# Autodesk Inventor assembly: GFRP_T2_01
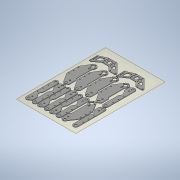
[picture p0: Inventor's stored thumbnail of the model, 180x180]
Saved by Autodesk Inventor 2020 (Build 240168000, 168)
## iProperties
Created: 2021-08-27
Part Number: GFRP_T2_01
Document SubType Name: Assembly
Designer: Masato
Author: Masato
## Documents named in this file (5)
- C:\Users\naoki\Documents\Inventor\CitBrains\git_clone\OpenPlatform4_1\GFRP\OpenPlatform_ver3_0\cam\GFRP_T2_01.iam
- C:\Users\naoki\Documents\Inventor\CitBrains\git_clone\OpenPlatform4_1\GFRP\OpenPlatform_ver3_0\cam\Disposable_Board.ipt
- C:\Users\naoki\Documents\Inventor\CitBrains\git_clone\OpenPlatform4_1\GFRP\OpenPlatform_ver3_0\LowerBody\Link\BackLink_frame.ipt
- C:\Users\naoki\Documents\Inventor\CitBrains\git_clone\OpenPlatform4_1\GFRP\OpenPlatform_ver3_0\LowerBody\Link\FrontLink_frame.ipt
- C:\Users\naoki\Documents\Inventor\CitBrains\git_clone\OpenPlatform4_1\GFRP\OpenPlatform_ver3_0\UpperBody\Head\Head_side_frame.ipt
## Components (16 placed, 4 different names)
1. Disposable_Board:1 — メイト:2, メイト:1, フラッシュ:1, フラッシュ:2, メイト:4, 正接:1, 正接:2, フラッシュ:5, フラッシュ:6, 角度:1, 正接:3, 正接:4, メイト:8, フラッシュ:11
2. BackLink_frame:7 — フラッシュ:8, フラッシュ:9, 角度:2, 正接:6, 正接:7
3. BackLink_frame:8 — フラッシュ:9, 角度:1, 角度:2, 正接:4, 正接:7, メイト:7
4. FrontLink_frame:5 — フラッシュ:10, メイト:6, 正接:3, 正接:5, メイト:7
5. BackLink_frame:1 — メイト:4, 正接:1, フラッシュ:4, メイト:5
6. BackLink_frame:2 — フラッシュ:4, メイト:5, 正接:2, フラッシュ:5, フラッシュ:7
7. BackLink_frame:3
8. BackLink_frame:4
9. BackLink_frame:5 — フラッシュ:10, メイト:6
10. BackLink_frame:6
11. FrontLink_frame:1 — フラッシュ:7, フラッシュ:6
12. FrontLink_frame:2 — 正接:8
13. FrontLink_frame:3
14. FrontLink_frame:4 — フラッシュ:8, 正接:5, 正接:6
15. Head_side_frame:1 — メイト:8, フラッシュ:11, 正接:8
16. Head_side_frame:2
## Component patterns: (3 elements, first: BackLink_frame:1 + BackLink_frame:2), (4 elements, first: FrontLink_frame:1), (2 elements, first: Head_side_frame:1)
## Relationships (27: Flush 10, Tangent 8, Mate 7, Angle 2)
- メイト:2 [Mate]: Disposable_Board:1
- メイト:1 [Mate]: Disposable_Board:1
- フラッシュ:1 [Flush]: Disposable_Board:1
- フラッシュ:2 [Flush]: Disposable_Board:1
- メイト:4 [Mate]: Disposable_Board:1 ↔ BackLink_frame:1
- 正接:1 [Tangent] (2 mm): Disposable_Board:1 ↔ BackLink_frame:1
- フラッシュ:4 [Flush]: BackLink_frame:1 ↔ BackLink_frame:2
- メイト:5 [Mate] (2.5 mm): BackLink_frame:1 ↔ BackLink_frame:2
- 正接:2 [Tangent] (2 mm): Disposable_Board:1 ↔ BackLink_frame:2
- フラッシュ:5 [Flush] (2 mm): Disposable_Board:1 ↔ BackLink_frame:2
- フラッシュ:7 [Flush]: BackLink_frame:2 ↔ FrontLink_frame:1
- フラッシュ:6 [Flush] (2 mm): Disposable_Board:1 ↔ FrontLink_frame:1
- フラッシュ:8 [Flush]: BackLink_frame:7 ↔ FrontLink_frame:4
- フラッシュ:9 [Flush]: BackLink_frame:7 ↔ BackLink_frame:8
- 角度:1 [Angle] (0 deg): Disposable_Board:1 ↔ BackLink_frame:8
- 角度:2 [Angle] (0 deg): BackLink_frame:7 ↔ BackLink_frame:8
- フラッシュ:10 [Flush]: FrontLink_frame:5 ↔ BackLink_frame:5
- メイト:6 [Mate] (2.5 mm): FrontLink_frame:5 ↔ BackLink_frame:5
- 正接:3 [Tangent] (2 mm): Disposable_Board:1 ↔ FrontLink_frame:5
- 正接:4 [Tangent] (2 mm): Disposable_Board:1 ↔ BackLink_frame:8
- 正接:5 [Tangent] (2.5 mm): FrontLink_frame:5 ↔ FrontLink_frame:4
- 正接:6 [Tangent] (2.5 mm): BackLink_frame:7 ↔ FrontLink_frame:4
- 正接:7 [Tangent] (2.5 mm): BackLink_frame:7 ↔ BackLink_frame:8
- メイト:7 [Mate] (2.5 mm): BackLink_frame:8 ↔ FrontLink_frame:5
- メイト:8 [Mate]: Disposable_Board:1 ↔ Head_side_frame:1
- フラッシュ:11 [Flush] (2 mm): Disposable_Board:1 ↔ Head_side_frame:1
- 正接:8 [Tangent] (2.5 mm): FrontLink_frame:2 ↔ Head_side_frame:1
